# Autodesk Inventor assembly: 4_Mecanum_Wheel_276-1447_MIR
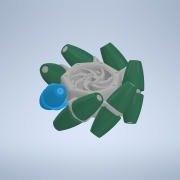
[picture p0: Inventor's stored thumbnail of the model, 180x180]
Saved by Autodesk Inventor 2020 (Build 240168000, 168)
## iProperties
Created: 2018-08-22
Part Number: 4_Mecanum_Wheel_276-1447_MIR
Material: 常规
Description: STEP AP214
Document SubType Name: Assembly
Designer: aresp
Sending System: SolidWorks 2017
Preprocessor: SwSTEP 2.0
Title: 217-1477-000 Rev3.STEP
Revision Number: ANY
## Documents named in this file (4)
- D:\Valut\ncrCadLib\轮子\4_Mecanum_Wheel_276-1447_MIR.iam
- D:\Valut\ncrCadLib\轮子\Components\276-1447-002 Rev3_MIR.ipt
- D:\Valut\ncrCadLib\轮子\Components\276-1447-001 Rev3_MIR.ipt
- D:\Valut\ncrCadLib\轮子\Components\276-1447-010 Rev1_MIR.iam
## Components (9 placed, 3 different names)
1. 276-1447-002 Rev3_MIR:1 — 配合:1
2. 276-1447-001 Rev3_MIR:1
3. 276-1447-010 Rev1_MIR:1 [sub-assembly]
4. 276-1447-010 Rev1_MIR:2 [sub-assembly]
5. 276-1447-010 Rev1_MIR:3 [sub-assembly]
6. 276-1447-010 Rev1_MIR:4 [sub-assembly]
7. 276-1447-010 Rev1_MIR:5 [sub-assembly]
8. 276-1447-010 Rev1_MIR:6 [sub-assembly]
9. 276-1447-010 Rev1_MIR:7 [sub-assembly]
## Relationships (1: Mate 1)
- 配合:1 [Mate]: 276-1447-002 Rev3_MIR:1
